# Autodesk Inventor assembly: button_box_assembly
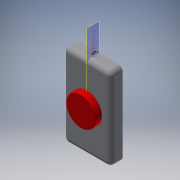
[picture p0: Inventor's stored thumbnail of the model, 180x180]
Saved by Autodesk Inventor 2016 (Build 200138000, 138)
## iProperties
Created: 2016-01-30
Part Number: button_box_assembly
Document SubType Name: Assembly
Designer: Greg
Author: Greg
## Documents named in this file (3)
- C:\Users\Greg\Desktop\PROJECTS\Programming\hackerman_2016\Inventor_Assets\button_box_assembly.iam
- C:\Users\Greg\Desktop\PROJECTS\Programming\hackerman_2016\Inventor_Assets\box_with_button.ipt
- C:\Users\Greg\Desktop\PROJECTS\Programming\hackerman_2016\Inventor_Assets\button_for_box.ipt
## Components (2 placed, 2 different names)
1. box_with_button:1 — Mate:1
2. button_for_box:1 — Mate:1
## Relationships (1: Mate 1)
- Mate:1: box_with_button:1 ↔ button_for_box:1
